# Autodesk Inventor assembly: SSE Ferula FO DC
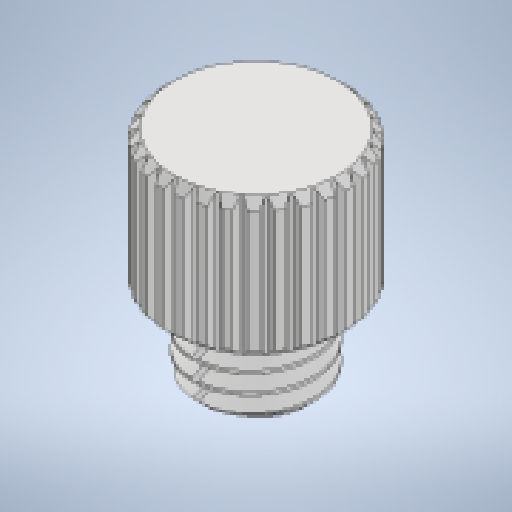
[picture p0: Inventor's stored thumbnail of the model, 512x512]
Saved by Autodesk Inventor 2024.2 (Build 282272000, 272)
## iProperties
Created: 2025-11-11
Part Number: SSE Ferula FO DC
Document SubType Name: Assembly
Designer: ja.restrepo1
Author: ja.restrepo1
## Documents named in this file (3)
- I:\MICROMECANICA\ALTAS ENERGIAS\Deteccion de Muones\Detectores centelladores\Partes Detector Centellador\SE Matriz Centelladora DC\Ferula Fiber Op\SSE Ferula FO DC.iam
- I:\MICROMECANICA\ALTAS ENERGIAS\Deteccion de Muones\Detectores centelladores\Partes Detector Centellador\SE Matriz Centelladora DC\Ferula Fiber Op\Ferula Optica.ipt
- I:\MICROMECANICA\ALTAS ENERGIAS\Deteccion de Muones\Detectores centelladores\Partes Detector Centellador\SE Matriz Centelladora DC\Ferula Fiber Op\Tuerca M12 2 IN.ipt
## Components (2 placed, 2 different names)
1. Ferula Optica:1 — Nivelación:1, Nivelación:2, Nivelación:3, Coincidencia:1, Coincidencia:2
2. Tuerca M12 2 IN:1 — Coincidencia:2
## Relationships (5: Flush 3, Mate 2)
- Nivelación:1 [Flush]: Ferula Optica:1
- Nivelación:2 [Flush]: Ferula Optica:1
- Nivelación:3 [Flush]: Ferula Optica:1
- Coincidencia:1 [Mate]: Ferula Optica:1
- Coincidencia:2 [Mate]: Ferula Optica:1 ↔ Tuerca M12 2 IN:1
